# Autodesk Inventor assembly: EBRI-10R
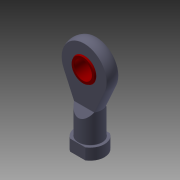
[picture p0: Inventor's stored thumbnail of the model, 180x180]
Saved by Autodesk Inventor 2016 SP1 (Build 200210100, 210)
## iProperties
Category: Bearing
Company: Autodesk, Inc.
Created: 2015-11-21
Part Number: EBRI-10R
Catalog Web Link: http://www.igus.com/iPro/iPro_02_0030_0000_USen.htm?c=US&l=en
Description: igubal Rod End Bearing
Vendor: igus
Document SubType Name: Assembly
Mass: 29.1846 g
Surface Area: 106.697 cm^2
Volume: 25.0095 cm^3
Density: 1.16694 g/cm^3
Project: FIRST
Engineer: Autodesk, Inc.
Title: igubal Rod End Bearing
Author: Autodesk, Inc.
Keywords: FIRSTChoice
## Documents named in this file (3)
- D:\FIRST\FRC KOP 2016\FRC FIRSTChoice 2016\fc16-057_RodEnd.iam
- D:\FIRST\FRC KOP 2016\FRC FIRSTChoice 2016\Parts\EBRI-10R_Housing.ipt
- D:\FIRST\FRC KOP 2016\FRC FIRSTChoice 2016\Parts\EBRI-10R_Spherical Bearing.ipt
## Components (2 placed, 2 different names)
1. EBRI-10R_Housing:1 — Mate:1, Angle:1
2. EBRI-10R_Spherical Bearing:1 — Mate:1, Angle:1
## Relationships (2: Mate 1, Angle 1)
- Mate:1: EBRI-10R_Housing:1 ↔ EBRI-10R_Spherical Bearing:1
- Angle:1 (0 deg): EBRI-10R_Housing:1 ↔ EBRI-10R_Spherical Bearing:1
